# Autodesk Inventor assembly: ShooterConceptA
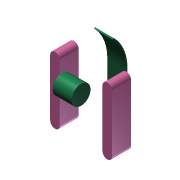
[picture p0: Inventor's stored thumbnail of the model, 180x180]
Saved by Autodesk Inventor 2012 (Build 160160000, 160)
## iProperties
Created: 2012-01-09
Part Number: ShooterConceptA
Document SubType Name: Assembly
Designer: JesseK
Author: JesseK
## Documents named in this file (3)
- Z:\UserData\Documents\Inventor\team1885frc\Robot2012\Concepts\ShooterConceptA.iam
- Z:\UserData\Documents\Inventor\team1885frc\Robot2012\Concepts\ShooterAcceleratorConcept.ipt
- Z:\UserData\Documents\Inventor\team1885frc\Robot2012\Concepts\ShooterWheelrConcept.ipt
## Components (3 placed, 2 different names)
1. ShooterAcceleratorConcept:1 — Mate:1, Mate:2, Flush:1, Mate:3
2. ShooterAcceleratorConcept:2 — Mate:1, Tangent:1, Flush:1
3. ShooterWheelrConcept:1 — Mate:2, Tangent:1, Mate:3
## Relationships (5: Mate 3, Tangent 1, Flush 1)
- Mate:1 (228.6 mm): ShooterAcceleratorConcept:1 ↔ ShooterAcceleratorConcept:2
- Mate:2 (63.5 mm): ShooterAcceleratorConcept:1 ↔ ShooterWheelrConcept:1
- Tangent:1: ShooterAcceleratorConcept:2 ↔ ShooterWheelrConcept:1
- Flush:1: ShooterAcceleratorConcept:1 ↔ ShooterAcceleratorConcept:2
- Mate:3: ShooterAcceleratorConcept:1 ↔ ShooterWheelrConcept:1
